# Autodesk Inventor assembly: Full box Corect
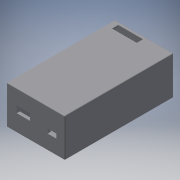
[picture p0: Inventor's stored thumbnail of the model, 180x180]
Saved by Autodesk Inventor 2019.3 (Build 233278000, 278)
## iProperties
Created: 2019-04-11
Part Number: Full box Corect
Document SubType Name: Assembly
Designer: grego
Author: grego
## Documents named in this file (4)
- D:\OneDrive - njit.edu\ECE 414-001\CAD model\Full box Corect.iam
- D:\OneDrive - njit.edu\ECE 414-001\CAD model\Half Box Correct.iam
- D:\OneDrive - njit.edu\ECE 414-001\CAD model\Smart Lock Box Top Correct.ipt
- Assembly1.ipt
## Components (2 placed, 2 different names)
1. Half Box Correct:1 [sub-assembly] — Flush:1, Flush:2, Flush:3, Flush:4, Flush:5, Mate:1
2. Smart Lock Box Top Correct:1 — Flush:1, Flush:2, Flush:3, Flush:4, Flush:5, Mate:1
## Relationships (6: Flush 5, Mate 1)
- Flush:1: Half Box Correct:1 ↔ Smart Lock Box Top Correct:1
- Flush:2: Half Box Correct:1 ↔ Smart Lock Box Top Correct:1
- Flush:3: Half Box Correct:1 ↔ Smart Lock Box Top Correct:1
- Flush:4: Half Box Correct:1 ↔ Smart Lock Box Top Correct:1
- Flush:5: Half Box Correct:1 ↔ Smart Lock Box Top Correct:1
- Mate:1: Half Box Correct:1 ↔ Smart Lock Box Top Correct:1
